# Autodesk Inventor assembly: Leg_joint_roll_pitch
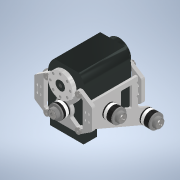
[picture p0: Inventor's stored thumbnail of the model, 180x180]
Saved by Autodesk Inventor 2020.4 (Build 244396000, 396)
## iProperties
Part Number: Leg_joint_roll_pitch
Document SubType Name: Assembly
Designer: Masato Kubotera
Mass: 155.537 g
Surface Area: 333.044 cm^2
Volume: 75.5065 cm^3
Density: 2.05992 g/cm^3
Author: Masato Kubotera
## Documents named in this file (16)
- C:\Users\Masato\Documents\Inventor\CIT Brains_Inventor\OpenPlatform_ver3_0\LowerBody\Leg_joit\Leg_joint_roll_pitch.iam
- C:\Users\Masato\Documents\Inventor\CIT Brains_Inventor\OpenPlatform_ver3_0\LowerBody\Leg_joit\Leg_joint_pitch_frame.ipt
- C:\Users\Masato\Documents\Inventor\CIT Brains_Inventor\OpenPlatform_ver3_0\LowerBody\Leg_joit\Leg_joint_roll_frame.ipt
- C:\Users\Masato\Documents\Inventor\CIT Brains_Inventor\OpenPlatform_ver3_0\Ready_Made\B3M11xx.ipt
- C:\Users\Masato\Documents\Inventor\CIT Brains_Inventor\OpenPlatform_ver3_0\Ready_Made\SLSBF6-39_5-M3-N3.ipt
- C:\Users\Masato\Documents\Inventor\CIT Brains_Inventor\OpenPlatform_ver3_0\Ready_Made\UUW-0312-10BH.ipt
- C:\Users\Masato\Documents\Inventor\CIT Brains_Inventor\OpenPlatform_ver3_0\Ready_Made\S3-07-3W.ipt
- C:\Users\Masato\Documents\Inventor\CIT Brains_Inventor\OpenPlatform_ver3_0\Ready_Made\CC-0612-25.ipt
- C:\Users\Masato\Documents\Inventor\CIT Brains_Inventor\OpenPlatform_ver3_0\Ready_Made\CC-0612-20B.ipt
- C:\Users\Masato\Documents\Inventor\CIT Brains_Inventor\OpenPlatform_ver3_0\Ready_Made\BRU-311S.ipt
- C:\Users\Masato\Documents\Inventor\CIT Brains_Inventor\OpenPlatform_ver3_0\Ready_Made\ARU-309S.ipt
- C:\Users\Masato\Documents\Inventor\CIT Brains_Inventor\OpenPlatform_ver3_0\Ready_Made\Screw\M3-6.ipt
- C:\Users\Masato\Documents\Inventor\CIT Brains_Inventor\OpenPlatform_ver3_0\Ready_Made\Screw\M2_6-20.ipt
- C:\Users\Masato\Documents\Inventor\CIT Brains_Inventor\OpenPlatform_ver3_0\Ready_Made\Screw\M2_6-15.ipt
- C:\Users\Masato\Documents\Inventor\CIT Brains_Inventor\OpenPlatform_ver3_0\Ready_Made\80F-0603.ipt
- C:\Users\Masato\Documents\Inventor\CIT Brains_Inventor\OpenPlatform_ver3_0\Ready_Made\free_horn.ipt
## Components (53 placed, 15 different names)
1. Leg_joint_pitch_frame:1 — メイト:2, フラッシュ:1, 挿入:11, 挿入:27, 挿入:28, 挿入:45
2. Leg_joint_pitch_frame:2 — メイト:3, メイト:4, フラッシュ:2, 挿入:12, 挿入:25, 挿入:26, 挿入:46, フラッシュ:1
3. Leg_joint_roll_frame:1 — 挿入:3, 挿入:4, 挿入:5, 挿入:6, メイト:2, メイト:3, メイト:4, フラッシュ:2, 挿入:81, 挿入:104, 挿入:106, 挿入:107, 挿入:108, 挿入:109
4. Leg_joint_roll_frame:2 — 挿入:7, 挿入:8, 挿入:9, 挿入:10, 挿入:55, 挿入:105, 挿入:110, 挿入:111, 挿入:112, 挿入:113
5. B3M11xx:1 — 挿入:3, 挿入:4, 挿入:5, 挿入:6, 挿入:7, 挿入:8, 挿入:9, 挿入:10, フラッシュ:6, メイト:8, メイト:10, 挿入:120
6. SLSBF6-39_5-M3-N3:1 — 挿入:11, 挿入:12
7. UUW-0312-10BH:1 — 挿入:27, 挿入:83, 挿入:100
8. UUW-0312-10BH:2 — 挿入:28, 挿入:82, 挿入:101
9. UUW-0312-10BH:3 — 挿入:25, 挿入:90, 挿入:99
10. UUW-0312-10BH:4 — 挿入:26, 挿入:93, 挿入:98
11. S3-07-3W:1 — 挿入:45
12. S3-07-3W:2 — 挿入:46
13. UUW-0312-10BH:5 — 挿入:55, 挿入:96, 挿入:103
14. UUW-0312-10BH:6 — 挿入:81, 挿入:84, 挿入:102
15. CC-0612-25:1 — 挿入:82, 挿入:88
16. CC-0612-25:2 — 挿入:83, 挿入:86
17. CC-0612-25:3 — 挿入:90, 挿入:91
18. CC-0612-25:4 — 挿入:93, 挿入:94
19. CC-0612-25:5 — 挿入:96, 挿入:97
20. CC-0612-25:6 — 挿入:84, 挿入:85
21. CC-0612-20B:1 — 挿入:88, 挿入:89
22. CC-0612-20B:2 — 挿入:86, 挿入:87
23. CC-0612-20B:3 — 挿入:85, 挿入:118
24. CC-0612-20B:4 — 挿入:92, 挿入:117
25. CC-0612-20B:5 — 挿入:94, 挿入:95
26. CC-0612-20B:6 — 挿入:97, 挿入:119
27. CC-0612-20B:7 — 挿入:89, 挿入:115
28. CC-0612-20B:8 — 挿入:87, 挿入:114
29. CC-0612-20B:9 — 挿入:91, 挿入:92
30. CC-0612-20B:10 — 挿入:95, 挿入:116
31. BRU-311S:1 — 挿入:99
32. BRU-311S:2 — 挿入:98
33. BRU-311S:3 — 挿入:101
34. BRU-311S:4 — 挿入:100
35. ARU-309S:1 — 挿入:102
36. ARU-309S:2 — 挿入:103
37. M3-6:1 — 挿入:104
38. M3-6:2 — 挿入:105
39. M2_6-20:1 — 挿入:106
40. M2_6-20:2 — 挿入:107
41. M2_6-20:3 — 挿入:108
42. M2_6-20:4 — 挿入:109
43. M2_6-15:1 — 挿入:110
44. M2_6-15:2 — 挿入:111
45. M2_6-15:3 — 挿入:112
46. M2_6-15:4 — 挿入:113
47. 80F-0603:1 — 挿入:118
48. 80F-0603:2 — 挿入:119
49. 80F-0603:3 — 挿入:114
50. 80F-0603:4 — 挿入:115
51. 80F-0603:5 — 挿入:117
52. 80F-0603:6 — 挿入:116
53. free_horn:1 — 挿入:120
## Relationships (65: Insert 57, Mate 5, Flush 3)
- 挿入:3 [Insert]: Leg_joint_roll_frame:1 ↔ B3M11xx:1
- 挿入:4 [Insert]: Leg_joint_roll_frame:1 ↔ B3M11xx:1
- 挿入:5 [Insert]: Leg_joint_roll_frame:1 ↔ B3M11xx:1
- 挿入:6 [Insert]: Leg_joint_roll_frame:1 ↔ B3M11xx:1
- 挿入:7 [Insert]: Leg_joint_roll_frame:2 ↔ B3M11xx:1
- 挿入:8 [Insert]: Leg_joint_roll_frame:2 ↔ B3M11xx:1
- 挿入:9 [Insert]: Leg_joint_roll_frame:2 ↔ B3M11xx:1
- 挿入:10 [Insert]: Leg_joint_roll_frame:2 ↔ B3M11xx:1
- メイト:2 [Mate] (0.01 mm): Leg_joint_pitch_frame:1 ↔ Leg_joint_roll_frame:1
- フラッシュ:1 [Flush]: Leg_joint_pitch_frame:1 ↔ Leg_joint_pitch_frame:2
- メイト:3 [Mate] (0.01 mm): Leg_joint_pitch_frame:2 ↔ Leg_joint_roll_frame:1
- メイト:4 [Mate] (0.01 mm): Leg_joint_pitch_frame:2 ↔ Leg_joint_roll_frame:1
- フラッシュ:2 [Flush]: Leg_joint_pitch_frame:2 ↔ Leg_joint_roll_frame:1
- 挿入:11 [Insert]: Leg_joint_pitch_frame:1 ↔ SLSBF6-39_5-M3-N3:1
- 挿入:12 [Insert]: Leg_joint_pitch_frame:2 ↔ SLSBF6-39_5-M3-N3:1
- 挿入:25 [Insert]: Leg_joint_pitch_frame:2 ↔ UUW-0312-10BH:3
- 挿入:26 [Insert]: Leg_joint_pitch_frame:2 ↔ UUW-0312-10BH:4
- 挿入:27 [Insert]: Leg_joint_pitch_frame:1 ↔ UUW-0312-10BH:1
- 挿入:28 [Insert]: Leg_joint_pitch_frame:1 ↔ UUW-0312-10BH:2
- フラッシュ:6 [Flush]: B3M11xx:1
- メイト:8 [Mate]: B3M11xx:1
- 挿入:45 [Insert]: Leg_joint_pitch_frame:1 ↔ S3-07-3W:1
- 挿入:46 [Insert]: Leg_joint_pitch_frame:2 ↔ S3-07-3W:2
- 挿入:55 [Insert]: Leg_joint_roll_frame:2 ↔ UUW-0312-10BH:5
- メイト:10 [Mate]: B3M11xx:1
- 挿入:81 [Insert]: Leg_joint_roll_frame:1 ↔ UUW-0312-10BH:6
- 挿入:82 [Insert]: UUW-0312-10BH:2 ↔ CC-0612-25:1
- 挿入:83 [Insert]: UUW-0312-10BH:1 ↔ CC-0612-25:2
- 挿入:84 [Insert]: UUW-0312-10BH:6 ↔ CC-0612-25:6
- 挿入:85 [Insert]: CC-0612-25:6 ↔ CC-0612-20B:3
- 挿入:86 [Insert]: CC-0612-25:2 ↔ CC-0612-20B:2
- 挿入:87 [Insert]: CC-0612-20B:2 ↔ CC-0612-20B:8
- 挿入:88 [Insert]: CC-0612-25:1 ↔ CC-0612-20B:1
- 挿入:89 [Insert]: CC-0612-20B:1 ↔ CC-0612-20B:7
- 挿入:90 [Insert]: UUW-0312-10BH:3 ↔ CC-0612-25:3
- 挿入:91 [Insert]: CC-0612-25:3 ↔ CC-0612-20B:9
- 挿入:92 [Insert]: CC-0612-20B:4 ↔ CC-0612-20B:9
- 挿入:93 [Insert]: UUW-0312-10BH:4 ↔ CC-0612-25:4
- 挿入:94 [Insert]: CC-0612-25:4 ↔ CC-0612-20B:5
- 挿入:95 [Insert]: CC-0612-20B:5 ↔ CC-0612-20B:10
- 挿入:96 [Insert]: UUW-0312-10BH:5 ↔ CC-0612-25:5
- 挿入:97 [Insert]: CC-0612-25:5 ↔ CC-0612-20B:6
- 挿入:98 [Insert]: UUW-0312-10BH:4 ↔ BRU-311S:2
- 挿入:99 [Insert]: UUW-0312-10BH:3 ↔ BRU-311S:1
- 挿入:100 [Insert]: UUW-0312-10BH:1 ↔ BRU-311S:4
- 挿入:101 [Insert]: UUW-0312-10BH:2 ↔ BRU-311S:3
- 挿入:102 [Insert]: UUW-0312-10BH:6 ↔ ARU-309S:1
- 挿入:103 [Insert]: UUW-0312-10BH:5 ↔ ARU-309S:2
- 挿入:104 [Insert]: Leg_joint_roll_frame:1 ↔ M3-6:1
- 挿入:105 [Insert]: Leg_joint_roll_frame:2 ↔ M3-6:2
- 挿入:106 [Insert]: Leg_joint_roll_frame:1 ↔ M2_6-20:1
- 挿入:107 [Insert]: Leg_joint_roll_frame:1 ↔ M2_6-20:2
- 挿入:108 [Insert]: Leg_joint_roll_frame:1 ↔ M2_6-20:3
- 挿入:109 [Insert]: Leg_joint_roll_frame:1 ↔ M2_6-20:4
- 挿入:110 [Insert]: Leg_joint_roll_frame:2 ↔ M2_6-15:1
- 挿入:111 [Insert]: Leg_joint_roll_frame:2 ↔ M2_6-15:2
- 挿入:112 [Insert]: Leg_joint_roll_frame:2 ↔ M2_6-15:3
- 挿入:113 [Insert]: Leg_joint_roll_frame:2 ↔ M2_6-15:4
- 挿入:114 [Insert]: CC-0612-20B:8 ↔ 80F-0603:3
- 挿入:115 [Insert]: CC-0612-20B:7 ↔ 80F-0603:4
- 挿入:116 [Insert]: CC-0612-20B:10 ↔ 80F-0603:6
- 挿入:117 [Insert]: CC-0612-20B:4 ↔ 80F-0603:5
- 挿入:118 [Insert]: CC-0612-20B:3 ↔ 80F-0603:1
- 挿入:119 [Insert]: CC-0612-20B:6 ↔ 80F-0603:2
- 挿入:120 [Insert]: B3M11xx:1 ↔ free_horn:1
